# Autodesk Inventor assembly: steering_hub_assembly
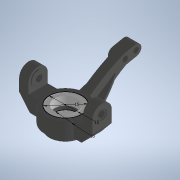
[picture p0: Inventor's stored thumbnail of the model, 180x180]
Saved by Autodesk Inventor 2020 (Build 240168000, 168)
## iProperties
Created: 2019-12-02
Part Number: steering_hub_assembly
Document SubType Name: Assembly
Designer: maste
Author: maste
## Documents named in this file (5)
- C:\Users\maste\Documents\GitHub\autobot\robot_model\steering_hub_assembly.iam
- C:\Users\maste\Documents\GitHub\autobot\robot_model\RCT-P006_steering_knuckle_OK.ipt
- C:\Users\maste\Documents\GitHub\autobot\robot_model\BR115ZZ.ipt
- C:\Users\maste\Documents\GitHub\autobot\robot_model\B6700ZZ.ipt
- C:\Users\maste\Documents\GitHub\autobot\robot_model\RCT-H019.ipt
## Components (5 placed, 4 different names)
1. RCT-P006_steering_knuckle_OK:1 — Mate:1, Flush:1, Mate:2, Flush:2, Mate:3, Mate:4, Mate:5, Mate:6
2. BR115ZZ:1 — Mate:1, Flush:1
3. B6700ZZ:1 — Mate:2, Flush:2
4. RCT-H019:1 — Mate:3, Mate:5
5. RCT-H019:2 — Mate:4, Mate:6
## Relationships (8: Mate 6, Flush 2)
- Mate:1: RCT-P006_steering_knuckle_OK:1 ↔ BR115ZZ:1
- Flush:1: RCT-P006_steering_knuckle_OK:1 ↔ BR115ZZ:1
- Mate:2: RCT-P006_steering_knuckle_OK:1 ↔ B6700ZZ:1
- Flush:2: RCT-P006_steering_knuckle_OK:1 ↔ B6700ZZ:1
- Mate:3: RCT-P006_steering_knuckle_OK:1 ↔ RCT-H019:1
- Mate:4: RCT-P006_steering_knuckle_OK:1 ↔ RCT-H019:2
- Mate:5: RCT-P006_steering_knuckle_OK:1 ↔ RCT-H019:1
- Mate:6: RCT-P006_steering_knuckle_OK:1 ↔ RCT-H019:2
